# Autodesk Inventor assembly: Assembly1
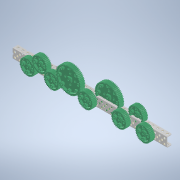
[picture p0: Inventor's stored thumbnail of the model, 180x180]
Saved by Autodesk Inventor 2022.2 (Build 262287010, 287A)
## iProperties
Created: 2022-05-21
Part Number: Assembly1
Document SubType Name: Assembly
Designer: Main Account
Author: Main Account
## Documents named in this file (10)
- D:\Documents\Inventor\VEX\Projects\TippingPointFinal\Assembly1.iam
- D:\Documents\Inventor\VEX\Library Backup\Library 1.3\Structure\C-Channels\Aluminum 1x2x1\Alu C 1x2x1x32.ipt
- D:\Documents\Inventor\VEX\Library Backup\Library 1.3\Motion\Gears\HS 60T Gear, Circle.ipt
- D:\Documents\Inventor\VEX\Library Backup\Library 1.3\Motion\Gears\HS 36T Gear, Circle.ipt
- D:\Documents\Inventor\VEX\Library Backup\Library 1.3\Structure\C-Channels\Aluminum 1x1 from VEX\Alu Half C VEX 1x1x3.ipt
- D:\Documents\Inventor\VEX\Library Backup\Library 1.3\Structure\C-Channels\Aluminum 1x1 from VEX\Alu Half C VEX 1x1x5.ipt
- D:\Documents\Inventor\VEX\Library Backup\Library 1.3\Motion\Spacers\Washer Steel\SWasher .375 OD x .031250.ipt
- D:\Documents\Inventor\VEX\Library Backup\Library 1.3\Motion\Spacers\Washer Steel.ipt
- D:\Documents\Inventor\VEX\Library Backup\Library 1.3\Motion\Spacers\Spacer Plastic\PSpacer 4.6.ipt
- D:\Documents\Inventor\VEX\Library Backup\Library 1.3\Motion\Spacers\Spacer Plastic.ipt
## Components (16 placed, 7 different names)
1. Alu C 1x2x1x32:1 — Insert:1, Insert:2, Insert:3, Insert:4, Insert:5, Mate:1, Mate:2, Mate:3, Mate:4, Insert:10, Insert:13
2. HS 60T Gear, Circle:1 — Insert:6
3. HS 60T Gear, Circle:2
4. HS 36T Gear, Circle:1 — Insert:1
5. HS 36T Gear, Circle:2 — Insert:4
6. HS 36T Gear, Circle:3 — Insert:3
7. HS 36T Gear, Circle:4 — Insert:2
8. HS 36T Gear, Circle:5 — Insert:5
9. HS 36T Gear, Circle:6 — Insert:7
10. HS 36T Gear, Circle:7
11. Alu Half C VEX 1x1x3:1 — Mate:1, Mate:2, Insert:7, Insert:8, Insert:9
12. Alu Half C VEX 1x1x5:1 — Mate:3, Mate:4, Insert:6, Insert:11, Insert:12
13. SWasher .375 OD x .031250:1 — Insert:8
14. SWasher .375 OD x .031250:2 — Insert:9, Insert:10
15. PSpacer 4.6:1 — Insert:11
16. PSpacer 4.6:2 — Insert:12, Insert:13
## Relationships (17: Insert 13, Mate 4)
- Insert:1: Alu C 1x2x1x32:1 ↔ HS 36T Gear, Circle:1
- Insert:2: Alu C 1x2x1x32:1 ↔ HS 36T Gear, Circle:4
- Insert:3: Alu C 1x2x1x32:1 ↔ HS 36T Gear, Circle:3
- Insert:4: Alu C 1x2x1x32:1 ↔ HS 36T Gear, Circle:2
- Insert:5: Alu C 1x2x1x32:1 ↔ HS 36T Gear, Circle:5
- Mate:1: Alu C 1x2x1x32:1 ↔ Alu Half C VEX 1x1x3:1
- Mate:2: Alu C 1x2x1x32:1 ↔ Alu Half C VEX 1x1x3:1
- Mate:3: Alu C 1x2x1x32:1 ↔ Alu Half C VEX 1x1x5:1
- Mate:4: Alu C 1x2x1x32:1 ↔ Alu Half C VEX 1x1x5:1
- Insert:6: HS 60T Gear, Circle:1 ↔ Alu Half C VEX 1x1x5:1
- Insert:7: HS 36T Gear, Circle:6 ↔ Alu Half C VEX 1x1x3:1
- Insert:8: Alu Half C VEX 1x1x3:1 ↔ SWasher .375 OD x .031250:1
- Insert:9: Alu Half C VEX 1x1x3:1 ↔ SWasher .375 OD x .031250:2
- Insert:10 (0.7937 mm): Alu C 1x2x1x32:1 ↔ SWasher .375 OD x .031250:2
- Insert:11: Alu Half C VEX 1x1x5:1 ↔ PSpacer 4.6:1
- Insert:12: Alu Half C VEX 1x1x5:1 ↔ PSpacer 4.6:2
- Insert:13: Alu C 1x2x1x32:1 ↔ PSpacer 4.6:2
